# Autodesk Inventor assembly: main_assembly
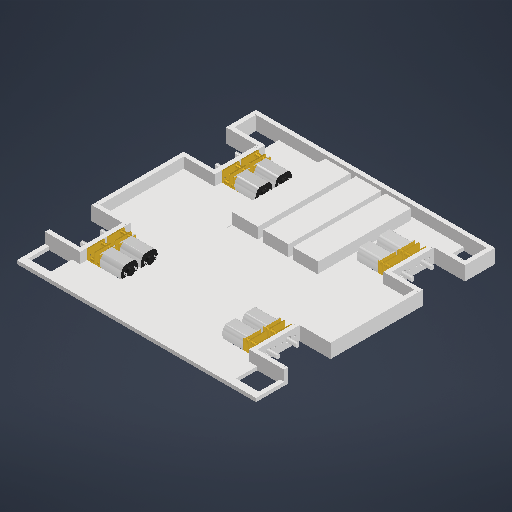
[picture p0: Inventor's stored thumbnail of the model, 512x512]
Saved by Autodesk Inventor 2026.2 (Build 302298010, 298A)
## iProperties
Created: 2026-03-12
Part Number: main_assembly
Document SubType Name: Assembly
Designer: karol
Author: karol
## Documents named in this file (16)
- C:\Users\karol\OneDrive\Desktop\robo\bolt\cad\assembly\main_assembly.iam
- C:\Users\karol\OneDrive\Desktop\robo\bolt\cad\assembly\base+motors.iam
- C:\Users\karol\OneDrive\Desktop\robo\bolt\cad\ready parts\backwall.ipt
- C:\Users\karol\OneDrive\Desktop\robo\bolt\cad\ready parts\left\left backside.ipt
- C:\Users\karol\OneDrive\Desktop\robo\bolt\cad\ready parts\right\right backside.ipt
- C:\Users\karol\OneDrive\Desktop\robo\bolt\cad\ready parts\right\roght backbackmotorwall.ipt
- C:\Users\karol\OneDrive\Desktop\robo\bolt\cad\ready parts\left\left backbackmotorwall.ipt
- C:\Users\karol\OneDrive\Desktop\robo\bolt\cad\ready parts\left\left back front motorwall; front, back and front motrowall.ipt
- C:\Users\karol\OneDrive\Desktop\robo\bolt\cad\ready parts\left\left sidewall.ipt
- C:\Users\karol\OneDrive\Desktop\robo\bolt\cad\ready parts\right\right back front motorwall; front, back and front motrowall.ipt
- C:\Users\karol\OneDrive\Desktop\robo\bolt\cad\ready parts\right\right sidewall.ipt
- C:\Users\karol\OneDrive\Desktop\robo\bolt\cad\ready parts\left\left frontfrontmotorwall.ipt
- C:\Users\karol\OneDrive\Desktop\robo\bolt\cad\ready parts\right\right frontfrontmotorwall.ipt
- C:\Users\karol\OneDrive\Desktop\robo\bolt\cad\ready parts\left\left insidemotorwall.ipt
- C:\Users\karol\OneDrive\Desktop\robo\bolt\cad\ready parts\right\right insidemotorwall.ipt
- C:\Users\karol\OneDrive\Desktop\robo\bolt\cad\ready parts\lipo.ipt
## Components (21 placed, 15 different names)
1. base+motors:1 [sub-assembly] — Mate:1, Mate:2, Mate:3, Mate:4, Mate:5, Mate:6, Mate:9, Mate:13, Mate:14, Mate:17, Mate:23, Mate:24, Mate:25, Mate:26, Mate:27, Mate:28, Mate:29, Mate:30, Mate:31, Mate:32, Mate:33, Mate:34, Mate:37, Mate:38, Mate:39, Mate:41, Mate:42, Mate:43, Mate:44, Mate:45, Mate:46, Mate:47, Mate:48, Mate:49, Mate:50
2. backwall:1 — Mate:1, Mate:2
3. left backside:1 — Mate:3, Mate:4, Mate:10
4. right backside:1 — Mate:5, Mate:6, Mate:35
5. left backbackmotorwall:1 — Mate:9, Mate:10
6. left back front motorwall; front, back and front motrowall:3 — Mate:13, Mate:14, Mate:18, Mate:40
7. left sidewall:1 — Mate:17, Mate:18
8. right back front motorwall; front, back and front motrowall:3 — Mate:23, Mate:24, Mate:36
9. right sidewall:1 — Mate:25, Mate:36
10. left frontfrontmotorwall:1 — Mate:28, Mate:29
11. left frontfrontmotorwall:2 — Mate:26, Mate:27
12. right frontfrontmotorwall:1 — Mate:30, Mate:31
13. right frontfrontmotorwall:2 — Mate:32, Mate:33
14. roght backbackmotorwall:1 — Mate:34, Mate:35
15. left insidemotorwall:1 — Mate:37, Mate:38
16. left insidemotorwall:2 — Mate:39, Mate:40
17. right insidemotorwall:1 — Mate:41, Mate:44
18. right insidemotorwall:2 — Mate:42, Mate:43
19. lipo:1 — Mate:49, Mate:50
20. lipo:2 — Mate:45, Mate:46
21. lipo:3 — Mate:47, Mate:48
## Relationships (40: Mate 40)
- Mate:1: base+motors:1 ↔ backwall:1
- Mate:2: base+motors:1 ↔ backwall:1
- Mate:3: base+motors:1 ↔ left backside:1
- Mate:4: base+motors:1 ↔ left backside:1
- Mate:5: base+motors:1 ↔ right backside:1
- Mate:6: base+motors:1 ↔ right backside:1
- Mate:9: base+motors:1 ↔ left backbackmotorwall:1
- Mate:10: left backside:1 ↔ left backbackmotorwall:1
- Mate:13: base+motors:1 ↔ left back front motorwall; front, back and front motrowall:3
- Mate:14: base+motors:1 ↔ left back front motorwall; front, back and front motrowall:3
- Mate:17: base+motors:1 ↔ left sidewall:1
- Mate:18: left back front motorwall; front, back and front motrowall:3 ↔ left sidewall:1
- Mate:23: base+motors:1 ↔ right back front motorwall; front, back and front motrowall:3
- Mate:24: base+motors:1 ↔ right back front motorwall; front, back and front motrowall:3
- Mate:25: base+motors:1 ↔ right sidewall:1
- Mate:26: base+motors:1 ↔ left frontfrontmotorwall:2
- Mate:27: base+motors:1 ↔ left frontfrontmotorwall:2
- Mate:28: base+motors:1 ↔ left frontfrontmotorwall:1
- Mate:29: base+motors:1 ↔ left frontfrontmotorwall:1
- Mate:30: base+motors:1 ↔ right frontfrontmotorwall:1
- Mate:31: base+motors:1 ↔ right frontfrontmotorwall:1
- Mate:32: base+motors:1 ↔ right frontfrontmotorwall:2
- Mate:33: base+motors:1 ↔ right frontfrontmotorwall:2
- Mate:34: base+motors:1 ↔ roght backbackmotorwall:1
- Mate:35: right backside:1 ↔ roght backbackmotorwall:1
- Mate:36: right back front motorwall; front, back and front motrowall:3 ↔ right sidewall:1
- Mate:37: base+motors:1 ↔ left insidemotorwall:1
- Mate:38: base+motors:1 ↔ left insidemotorwall:1
- Mate:39: base+motors:1 ↔ left insidemotorwall:2
- Mate:40: left back front motorwall; front, back and front motrowall:3 ↔ left insidemotorwall:2
- Mate:41: base+motors:1 ↔ right insidemotorwall:1
- Mate:42: base+motors:1 ↔ right insidemotorwall:2
- Mate:43: base+motors:1 ↔ right insidemotorwall:2
- Mate:44: base+motors:1 ↔ right insidemotorwall:1
- Mate:45: base+motors:1 ↔ lipo:2
- Mate:46: base+motors:1 ↔ lipo:2
- Mate:47: base+motors:1 ↔ lipo:3
- Mate:48: base+motors:1 ↔ lipo:3
- Mate:49: base+motors:1 ↔ lipo:1
- Mate:50: base+motors:1 ↔ lipo:1
